# Autodesk Inventor assembly: Pancake_Timing Assy_Lever Shaft
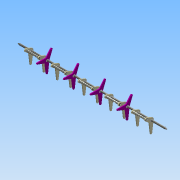
[picture p0: Inventor's stored thumbnail of the model, 180x180]
Saved by Autodesk Inventor 2018.1 (Build 221171000, 171)
## iProperties
Created: 2019-02-11
Part Number: Pancake_Timing Assy_Lever Shaft
Document SubType Name: Assembly
Designer: James
Author: James
## Documents named in this file (8)
- C:\Users\admin\Desktop\Ball Sorting Machine\Ball-Sorting-Machine\Pancake Sort\Pancake_Timing Assy_Lever Shaft.iam
- C:\Users\admin\Desktop\Ball Sorting Machine\Ball-Sorting-Machine\Timing Gate\Timing_Lever.ipt
- C:\Users\admin\Desktop\Ball Sorting Machine\Ball-Sorting-Machine\Pancake Sort\BS 3673 - 6mm External Circlip.ipt
- C:\Users\admin\Desktop\Ball Sorting Machine\Ball-Sorting-Machine\Timing Gate\M3 x 0.5mm Zinc Plated Steel Washer.ipt
- C:\Users\admin\Desktop\Ball Sorting Machine\Ball-Sorting-Machine\Timing Gate\Socket Button Head - (A2) - M3 x 10.ipt
- C:\Users\admin\Desktop\Ball Sorting Machine\Ball-Sorting-Machine\Pancake Sort\Pancake_Lever Shaft.ipt
- C:\Users\admin\Desktop\Ball Sorting Machine\Ball-Sorting-Machine\Pancake Sort\Pancake_Lever Weight.ipt
- C:\Users\admin\Desktop\Ball Sorting Machine\Ball-Sorting-Machine\Pancake Sort\Pancake_Switch Lever 2.ipt
## Components (68 placed, 7 different names)
1. Pancake_Lever Shaft:1 — Mate:45, Flush:18, Mate:46, Mate:47, Mate:48, Mate:49, Mate:56, Mate:62, Mate:63, Mate:64, Mate:65, Mate:66
2. BS 3673 - 6mm External Circlip:2 — Flush:10, Angle:2, Mate:47, Mate:48, Flush:19
3. BS 3673 - 6mm External Circlip:1 — Flush:10, Mate:46, Mate:49, Flush:19, Angle:3
4. BS 3673 - 6mm External Circlip:3 — Mate:61, Flush:20
5. BS 3673 - 6mm External Circlip:4
6. BS 3673 - 6mm External Circlip:5
7. BS 3673 - 6mm External Circlip:6
8. BS 3673 - 6mm External Circlip:7
9. BS 3673 - 6mm External Circlip:8
10. BS 3673 - 6mm External Circlip:9
11. BS 3673 - 6mm External Circlip:10
12. BS 3673 - 6mm External Circlip:11
13. BS 3673 - 6mm External Circlip:12
14. BS 3673 - 6mm External Circlip:13
15. BS 3673 - 6mm External Circlip:14
16. BS 3673 - 6mm External Circlip:15
17. BS 3673 - 6mm External Circlip:16
18. BS 3673 - 6mm External Circlip:17
19. BS 3673 - 6mm External Circlip:18
20. BS 3673 - 6mm External Circlip:19
21. BS 3673 - 6mm External Circlip:20
22. Socket Button Head - (A2) - M3 x 10:1 — Mate:15, Mate:16
23. M3 x 0.5mm Zinc Plated Steel Washer:1 — Mate:13, Mate:14, Mate:15
24. Timing_Lever:1 — Mate:7, Mate:8, Mate:13, Mate:14, Mate:16, Mate:45, Flush:18, Angle:4
25. Pancake_Lever Weight:1 — Mate:7, Mate:8, Mate:59, Mate:60
26. Socket Button Head - (A2) - M3 x 10:2 — Mate:52, Mate:54
27. M3 x 0.5mm Zinc Plated Steel Washer:2 — Mate:54, Mate:55
28. Timing_Lever:7 — Mate:56, Mate:59, Mate:52, Mate:55, Mate:60, Mate:61, Flush:22
29. Socket Button Head - (A2) - M3 x 10:3
30. M3 x 0.5mm Zinc Plated Steel Washer:3
31. Timing_Lever:2
32. Pancake_Lever Weight:2
33. Socket Button Head - (A2) - M3 x 10:4
34. M3 x 0.5mm Zinc Plated Steel Washer:4
35. Timing_Lever:8
36. Socket Button Head - (A2) - M3 x 10:5
37. M3 x 0.5mm Zinc Plated Steel Washer:5
38. Timing_Lever:3
39. Pancake_Lever Weight:3
40. Socket Button Head - (A2) - M3 x 10:6
41. M3 x 0.5mm Zinc Plated Steel Washer:6
42. Timing_Lever:9
43. Socket Button Head - (A2) - M3 x 10:7
44. M3 x 0.5mm Zinc Plated Steel Washer:7
45. Timing_Lever:4
46. Pancake_Lever Weight:4
47. Socket Button Head - (A2) - M3 x 10:8
48. M3 x 0.5mm Zinc Plated Steel Washer:8
49. Timing_Lever:10
50. Socket Button Head - (A2) - M3 x 10:9
51. M3 x 0.5mm Zinc Plated Steel Washer:9
52. Timing_Lever:5
53. Pancake_Lever Weight:5
54. Socket Button Head - (A2) - M3 x 10:10
55. M3 x 0.5mm Zinc Plated Steel Washer:10
56. Timing_Lever:11
57. BS 3673 - 6mm External Circlip:22 — Mate:62, Mate:65, Flush:20, Flush:21, Mate:67
58. Pancake_Switch Lever 2:1 — Mate:66, Mate:67, Flush:22
59. BS 3673 - 6mm External Circlip:21 — Mate:63, Mate:64, Flush:21
60. BS 3673 - 6mm External Circlip:23
61. Pancake_Switch Lever 2:2
62. BS 3673 - 6mm External Circlip:24
63. BS 3673 - 6mm External Circlip:25
64. Pancake_Switch Lever 2:3
65. BS 3673 - 6mm External Circlip:26
66. BS 3673 - 6mm External Circlip:27
67. Pancake_Switch Lever 2:4
68. BS 3673 - 6mm External Circlip:28
## Component patterns: (10 elements, first: BS 3673 - 6mm External Circlip:2 + BS 3673 - 6mm External Circlip:1), (5 elements, first: Socket Button Head - (A2) - M3 x 10:1 + M3 x 0.5mm Zinc Plated Steel Washer:1 + Timing_Lever:1 + Pancake_Lever Weight:1 + Socket Button Head - (A2) - M3 x 10:2 + M3 x 0.5mm Zinc Plated Steel Washer:2 + Timing_Lever:7), (4 elements, first: BS 3673 - 6mm External Circlip:22 + Pancake_Switch Lever 2:1 + BS 3673 - 6mm External Circlip:21)
## Relationships (40: Mate 25, Flush 12, Angle 3)
- [Flush]: Pancake_Lever Shaft:1
- Mate:7: Timing_Lever:1 ↔ Pancake_Lever Weight:1
- Mate:8: Timing_Lever:1 ↔ Pancake_Lever Weight:1
- Flush:10: BS 3673 - 6mm External Circlip:2 ↔ BS 3673 - 6mm External Circlip:1
- Angle:2 (180 deg): BS 3673 - 6mm External Circlip:2
- Mate:13: M3 x 0.5mm Zinc Plated Steel Washer:1 ↔ Timing_Lever:1
- Mate:14: M3 x 0.5mm Zinc Plated Steel Washer:1 ↔ Timing_Lever:1
- Mate:15: Socket Button Head - (A2) - M3 x 10:1 ↔ M3 x 0.5mm Zinc Plated Steel Washer:1
- Mate:16: Socket Button Head - (A2) - M3 x 10:1 ↔ Timing_Lever:1
- Flush:11 (-58 mm)
- Flush:12 (-5 mm)
- Flush:13 (30 mm)
- [Flush]: Pancake_Lever Shaft:1
- [Flush]: Pancake_Lever Shaft:1
- Mate:45: Pancake_Lever Shaft:1 ↔ Timing_Lever:1
- Flush:18: Pancake_Lever Shaft:1 ↔ Timing_Lever:1
- Mate:46: Pancake_Lever Shaft:1 ↔ BS 3673 - 6mm External Circlip:1
- Mate:47: Pancake_Lever Shaft:1 ↔ BS 3673 - 6mm External Circlip:2
- Mate:48: Pancake_Lever Shaft:1 ↔ BS 3673 - 6mm External Circlip:2
- Mate:49: Pancake_Lever Shaft:1 ↔ BS 3673 - 6mm External Circlip:1
- Flush:19: BS 3673 - 6mm External Circlip:2 ↔ BS 3673 - 6mm External Circlip:1
- Angle:3 (0 deg): BS 3673 - 6mm External Circlip:1
- [Mate]: Socket Button Head - (A2) - M3 x 10:2 ↔ M3 x 0.5mm Zinc Plated Steel Washer:2
- Mate:52: Socket Button Head - (A2) - M3 x 10:2 ↔ Timing_Lever:7
- Mate:54: Socket Button Head - (A2) - M3 x 10:2 ↔ M3 x 0.5mm Zinc Plated Steel Washer:2
- Mate:55: M3 x 0.5mm Zinc Plated Steel Washer:2 ↔ Timing_Lever:7
- Mate:56: Pancake_Lever Shaft:1 ↔ Timing_Lever:7
- Mate:59: Pancake_Lever Weight:1 ↔ Timing_Lever:7
- Mate:60: Pancake_Lever Weight:1 ↔ Timing_Lever:7
- Mate:61: BS 3673 - 6mm External Circlip:3 ↔ Timing_Lever:7
- Angle:4 (7.5 deg): Timing_Lever:1
- Mate:62: Pancake_Lever Shaft:1 ↔ BS 3673 - 6mm External Circlip:22
- Mate:63: Pancake_Lever Shaft:1 ↔ BS 3673 - 6mm External Circlip:21
- Mate:64: Pancake_Lever Shaft:1 ↔ BS 3673 - 6mm External Circlip:21
- Mate:65: Pancake_Lever Shaft:1 ↔ BS 3673 - 6mm External Circlip:22
- Flush:20: BS 3673 - 6mm External Circlip:3 ↔ BS 3673 - 6mm External Circlip:22
- Flush:21: BS 3673 - 6mm External Circlip:22 ↔ BS 3673 - 6mm External Circlip:21
- Mate:66: Pancake_Lever Shaft:1 ↔ Pancake_Switch Lever 2:1
- Mate:67: BS 3673 - 6mm External Circlip:22 ↔ Pancake_Switch Lever 2:1
- Flush:22: Timing_Lever:7 ↔ Pancake_Switch Lever 2:1
## Named parameters: d204_d35 = 0 mm
